# Autodesk Inventor assembly: 25197-02
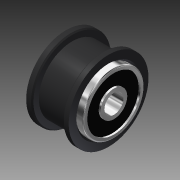
[picture p0: Inventor's stored thumbnail of the model, 180x180]
Saved by Autodesk Inventor 2014 (Build 180170000, 170)
## iProperties
Created: 2012-01-24
Part Number: 25197-02
Document SubType Name: Assembly
Designer: ERF
Catalog Web Link: varies
Description: Smooth Idler Assembly
Vendor: custom
Stock Number: B30041_ASM
Mass: 2.21849 g
Surface Area: 41.2914 cm^2
Volume: 1.85724 cm^3
Density: 1.19451 g/cm^3
Project: Shapeoko
User Status: F
Author: ERF
Subject: Motion
Title: Smooth Idler Assembly
## Documents named in this file (4)
- C:\Users\Edward\Documents\GitHub\Shapeoko_2\Autodesk_Inventor_Project\25197-02.iam
- C:\Users\Edward\Documents\GitHub\Shapeoko_2\Autodesk_Inventor_Project\25196-01.ipt
- C:\Users\Edward\Documents\GitHub\Shapeoko_2\Autodesk_Inventor_Project\25201-01.ipt
- C:\Users\Edward\Documents\GitHub\Shapeoko_2\Autodesk_Inventor_Project\25197-01.ipt
## Components (4 placed, 3 different names)
1. 25201-01:2 — Insert:2, Insert:3
2. 25196-01:3 — Insert:3
3. 25196-01:4 — Insert:1, Insert:2
4. 25197-01:2 — Insert:1
## Relationships (3: Insert 3)
- Insert:1: 25196-01:4 ↔ 25197-01:2
- Insert:2: 25201-01:2 ↔ 25196-01:4
- Insert:3: 25201-01:2 ↔ 25196-01:3
